# Autodesk Inventor assembly: bls-50-ac-adapter
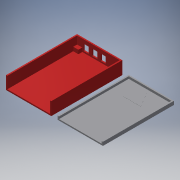
[picture p0: Inventor's stored thumbnail of the model, 180x180]
Saved by Autodesk Inventor 2017 (Build 210142000, 142)
## iProperties
Created: 2017-05-03
Part Number: bls-50-ac-adapter
Document SubType Name: Assembly
Designer: caleb
Author: caleb
## Documents named in this file (3)
- C:\cygwin64\home\caleb\olympus-bls-50-ac-adapter\bls-50-ac-adapter.iam
- C:\cygwin64\home\caleb\olympus-bls-50-ac-adapter\top.ipt
- C:\cygwin64\home\caleb\olympus-bls-50-ac-adapter\bottom.ipt
## Components (2 placed, 2 different names)
1. top:1 — Flush:1, Flush:2, Mate:1
2. bottom:1 — Flush:1, Flush:2, Mate:1
## Relationships (3: Flush 2, Mate 1)
- Flush:1: top:1 ↔ bottom:1
- Flush:2: top:1 ↔ bottom:1
- Mate:1 (5 mm): top:1 ↔ bottom:1
